# Autodesk Inventor assembly: 2016_IEEE_SouteastCon_Court v2
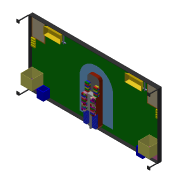
[picture p0: Inventor's stored thumbnail of the model, 180x180]
Saved by Autodesk Inventor 2015 (Build 190159000, 159)
## iProperties
Created: 2015-03-03
Part Number: 2016_IEEE_SouteastCon_Court v2
Document SubType Name: Assembly
Designer: Vukica
Author: Vukica
## Documents named in this file (17)
- C:\Users\Vukica\Dropbox\IEEE\hardware rules\2016Hardware_Court_v3\2016_IEEE_SouteastCon_Court v2.iam
- C:\Users\Vukica\Dropbox\IEEE\hardware rules\2016Hardware_Court\Base.ipt
- C:\Users\Vukica\Dropbox\IEEE\hardware rules\2016Hardware_Court\Ship area.ipt
- C:\Users\Vukica\Dropbox\IEEE\hardware rules\2016Hardware_Court\Starting position pink.ipt
- C:\Users\Vukica\Dropbox\IEEE\hardware rules\2016Hardware_Court\Starting position purple.ipt
- C:\Users\Vukica\Dropbox\IEEE\hardware rules\2016Hardware_Court\Rail zone.ipt
- C:\Users\Vukica\Dropbox\IEEE\hardware rules\2016Hardware_Court\Beacon.ipt
- C:\Users\Vukica\Dropbox\IEEE\hardware rules\2016Hardware_Court\Side 84 in by 6 in by half inch.ipt
- C:\Users\Vukica\Dropbox\IEEE\hardware rules\2016Hardware_Court\Side 120 in by 6 in by half inch.ipt
- C:\Users\Vukica\Dropbox\IEEE\hardware rules\2016Hardware_Court\Hill.ipt
- C:\Users\Vukica\Dropbox\IEEE\hardware rules\2016Hardware_Court\Blue truck.ipt
- C:\Users\Vukica\Dropbox\IEEE\hardware rules\2016Hardware_Court\Gold bar.ipt
- C:\Users\Vukica\Dropbox\IEEE\hardware rules\2016Hardware_Court\Tunnel.ipt
- C:\Users\Vukica\Dropbox\IEEE\hardware rules\2016Hardware_Court\Rail car.ipt
- C:\Users\Vukica\Dropbox\IEEE\hardware rules\2016Hardware_Court\Shipping goods QR subassembly.iam
- C:\Users\Vukica\Dropbox\IEEE\hardware rules\2016Hardware_Court\Shipping goods generic subassembly.iam
- C:\Users\Vukica\Dropbox\IEEE\hardware rules\2016Hardware_Court\Shipping goods colors subassembly.iam
## Components (36 placed, 16 different names)
1. Base:1 — Mate:1, Flush:1, Flush:2, Mate:2, Flush:3, Flush:4, Mate:3, Flush:5, Flush:6, Mate:4, Flush:7, Flush:8, Mate:5, Flush:9, Mate:7, Flush:11, Mate:9, Flush:12, Flush:13, Flush:15, Mate:10, Mate:11, Flush:16, Flush:18, Mate:12, Mate:17, Mate:22, Mate:30, Mate:38, Mate:40, Mate:43, Mate:46, Mate:53, Mate:55, Mate:62
2. Ship area:1 — Mate:1, Flush:1, Flush:2, Mate:6, Mate:49
3. Ship area:2 — Mate:2, Flush:3, Flush:4, Mate:8, Flush:10, Mate:54
4. Starting position pink:1 — Mate:4, Flush:7, Flush:8, Mate:64, Mate:88
5. Starting position purple:1 — Mate:3, Flush:5, Flush:6, Mate:89, Mate:105
6. Rail zone:1 — Mate:5, Mate:6, Flush:9, Mate:92, Flush:41
7. Rail zone:2 — Mate:7, Mate:8, Flush:10, Mate:90, Flush:40
8. Beacon:1 — Mate:14, Flush:22, Flush:23
9. Beacon:2 — Mate:13, Flush:20, Flush:21
10. Beacon:3 — Mate:15, Flush:24, Flush:25
11. Beacon:4 — Mate:16, Flush:26, Flush:27
12. Side 84 in by 6 in by half inch:1 — Mate:11, Flush:16, Flush:17, Mate:15, Flush:25, Mate:16, Flush:26, Flush:27, Mate:63, Flush:51
13. Side 84 in by 6 in by half inch:2 — Flush:18, Mate:12, Flush:19, Mate:13, Flush:21, Mate:14, Flush:23, Mate:39, Mate:41, Mate:44, Mate:47, Mate:106
14. Side 120 in by 6 in by half inch:1 — Flush:13, Flush:15, Mate:10, Flush:17, Flush:22, Flush:24, Mate:91, Mate:93
15. Side 120 in by 6 in by half inch:2 — Flush:11, Mate:9, Flush:12, Flush:19, Flush:20, Mate:23, Mate:32, Mate:84
16. Barge:1 — Mate:17, Mate:84, Mate:94, Flush:43, Flush:44, Mate:95, Flush:45, Flush:46, Mate:96, Mate:97, Flush:47, Mate:98, Flush:48, Mate:99, Mate:100, Flush:49, Mate:101, Mate:102, Flush:50, Mate:103, Flush:51
17. Blue truck:1 — Mate:22, Mate:23, Mate:89
18. Blue truck:2 — Mate:30, Mate:32, Mate:88
19. Gold bar:1 — Mate:38, Mate:39, Mate:42, Mate:45
20. Gold bar:2 — Mate:40, Mate:41, Mate:42, Mate:49
21. Gold bar:3 — Mate:43, Mate:44, Mate:45, Mate:48
22. Gold bar:4 — Mate:46, Mate:47, Mate:48
23. Gold bar:5 — Flush:30, Mate:50, Flush:31, Mate:51, Flush:32, Flush:33, Mate:53
24. Gold bar:6 — Flush:30, Mate:50, Flush:31, Mate:54, Mate:55
25. Gold bar:7 — Mate:51, Flush:32, Flush:33, Flush:34, Mate:52, Flush:35
26. Gold bar:8 — Flush:34, Mate:52, Flush:35
27. Tunnel:1 — Mate:62, Mate:63, Mate:64
28. Rail car:1 — Mate:90, Mate:91, Flush:40
29. Rail car:2 — Mate:92, Mate:93, Flush:41
30. Shipping goods QR subassembly:1 [sub-assembly] — Mate:94, Flush:43, Flush:44
31. Shipping goods QR subassembly:2 [sub-assembly] — Mate:95, Flush:45, Flush:46
32. Shipping goods generic subassembly:1 [sub-assembly] — Mate:96, Mate:97, Flush:47
33. Shipping goods generic subassembly:2 [sub-assembly] — Mate:98, Flush:48, Mate:99
34. Shipping goods colors subassembly:1 [sub-assembly] — Mate:102, Flush:50, Mate:103
35. Shipping goods colors subassembly:2 [sub-assembly] — Mate:100, Flush:49, Mate:101
36. Tunnel:2 — Mate:105, Mate:106
## Relationships (104: Mate 61, Flush 43)
- Mate:1: Base:1 ↔ Ship area:1
- Flush:1: Base:1 ↔ Ship area:1
- Flush:2: Base:1 ↔ Ship area:1
- Mate:2: Base:1 ↔ Ship area:2
- Flush:3: Base:1 ↔ Ship area:2
- Flush:4: Base:1 ↔ Ship area:2
- Mate:3: Base:1 ↔ Starting position purple:1
- Flush:5: Base:1 ↔ Starting position purple:1
- Flush:6: Base:1 ↔ Starting position purple:1
- Mate:4: Base:1 ↔ Starting position pink:1
- Flush:7: Base:1 ↔ Starting position pink:1
- Flush:8: Base:1 ↔ Starting position pink:1
- Mate:5: Base:1 ↔ Rail zone:1
- Mate:6: Ship area:1 ↔ Rail zone:1
- Flush:9: Base:1 ↔ Rail zone:1
- Mate:7: Base:1 ↔ Rail zone:2
- Mate:8: Ship area:2 ↔ Rail zone:2
- Flush:10: Ship area:2 ↔ Rail zone:2
- Flush:11: Base:1 ↔ Side 120 in by 6 in by half inch:2
- Mate:9: Base:1 ↔ Side 120 in by 6 in by half inch:2
- Flush:12: Base:1 ↔ Side 120 in by 6 in by half inch:2
- Flush:13: Base:1 ↔ Side 120 in by 6 in by half inch:1
- Flush:15: Base:1 ↔ Side 120 in by 6 in by half inch:1
- Mate:10: Base:1 ↔ Side 120 in by 6 in by half inch:1
- Mate:11: Base:1 ↔ Side 84 in by 6 in by half inch:1
- Flush:16: Base:1 ↔ Side 84 in by 6 in by half inch:1
- Flush:17: Side 84 in by 6 in by half inch:1 ↔ Side 120 in by 6 in by half inch:1
- Flush:18: Base:1 ↔ Side 84 in by 6 in by half inch:2
- Mate:12: Base:1 ↔ Side 84 in by 6 in by half inch:2
- Flush:19: Side 84 in by 6 in by half inch:2 ↔ Side 120 in by 6 in by half inch:2
- Mate:13: Beacon:2 ↔ Side 84 in by 6 in by half inch:2
- Flush:20: Beacon:2 ↔ Side 120 in by 6 in by half inch:2
- Flush:21: Beacon:2 ↔ Side 84 in by 6 in by half inch:2
- Mate:14: Beacon:1 ↔ Side 84 in by 6 in by half inch:2
- Flush:22: Beacon:1 ↔ Side 120 in by 6 in by half inch:1
- Flush:23: Beacon:1 ↔ Side 84 in by 6 in by half inch:2
- Mate:15: Beacon:3 ↔ Side 84 in by 6 in by half inch:1
- Flush:24: Beacon:3 ↔ Side 120 in by 6 in by half inch:1
- Flush:25: Beacon:3 ↔ Side 84 in by 6 in by half inch:1
- Mate:16: Beacon:4 ↔ Side 84 in by 6 in by half inch:1
- Flush:26: Beacon:4 ↔ Side 84 in by 6 in by half inch:1
- Flush:27: Beacon:4 ↔ Side 84 in by 6 in by half inch:1
- Mate:17: Base:1 ↔ Barge:1
- Mate:22: Base:1 ↔ Blue truck:1
- Mate:23: Side 120 in by 6 in by half inch:2 ↔ Blue truck:1
- Mate:30: Base:1 ↔ Blue truck:2
- Mate:32: Side 120 in by 6 in by half inch:2 ↔ Blue truck:2
- Mate:38: Base:1 ↔ Gold bar:1
- Mate:39: Side 84 in by 6 in by half inch:2 ↔ Gold bar:1
- Mate:40: Base:1 ↔ Gold bar:2
- Mate:41: Side 84 in by 6 in by half inch:2 ↔ Gold bar:2
- Mate:42: Gold bar:1 ↔ Gold bar:2
- Mate:43: Base:1 ↔ Gold bar:3
- Mate:44: Side 84 in by 6 in by half inch:2 ↔ Gold bar:3
- Mate:45: Gold bar:1 ↔ Gold bar:3
- Mate:46: Base:1 ↔ Gold bar:4
- Mate:47: Side 84 in by 6 in by half inch:2 ↔ Gold bar:4
- Mate:48: Gold bar:3 ↔ Gold bar:4
- Mate:49: Ship area:1 ↔ Gold bar:2
- Flush:30: Gold bar:5 ↔ Gold bar:6
- Mate:50: Gold bar:5 ↔ Gold bar:6
- Flush:31: Gold bar:5 ↔ Gold bar:6
- Mate:51: Gold bar:5 ↔ Gold bar:7
- Flush:32: Gold bar:5 ↔ Gold bar:7
- Flush:33: Gold bar:5 ↔ Gold bar:7
- Flush:34: Gold bar:7 ↔ Gold bar:8
- Mate:52: Gold bar:7 ↔ Gold bar:8
- Flush:35: Gold bar:7 ↔ Gold bar:8
- Mate:53: Base:1 ↔ Gold bar:5
- Mate:54: Ship area:2 ↔ Gold bar:6
- Mate:55: Base:1 ↔ Gold bar:6
- Mate:62: Base:1 ↔ Tunnel:1
- Mate:63: Side 84 in by 6 in by half inch:1 ↔ Tunnel:1
- Mate:64: Starting position pink:1 ↔ Tunnel:1
- Mate:84: Side 120 in by 6 in by half inch:2 ↔ Barge:1
- Mate:88: Starting position pink:1 ↔ Blue truck:2
- Mate:89: Starting position purple:1 ↔ Blue truck:1
- Mate:90: Rail zone:2 ↔ Rail car:1
- Mate:91 (50.8 mm): Side 120 in by 6 in by half inch:1 ↔ Rail car:1
- Flush:40: Rail zone:2 ↔ Rail car:1
- Mate:92: Rail zone:1 ↔ Rail car:2
- Mate:93 (50.8 mm): Side 120 in by 6 in by half inch:1 ↔ Rail car:2
- Flush:41: Rail zone:1 ↔ Rail car:2
- Mate:94: Barge:1 ↔ Shipping goods QR subassembly:1
- Flush:43: Barge:1 ↔ Shipping goods QR subassembly:1
- Flush:44: Barge:1 ↔ Shipping goods QR subassembly:1
- Mate:95: Barge:1 ↔ Shipping goods QR subassembly:2
- Flush:45: Barge:1 ↔ Shipping goods QR subassembly:2
- Flush:46: Barge:1 ↔ Shipping goods QR subassembly:2
- Mate:96: Barge:1 ↔ Shipping goods generic subassembly:1
- Mate:97: Barge:1 ↔ Shipping goods generic subassembly:1
- Flush:47: Barge:1 ↔ Shipping goods generic subassembly:1
- Mate:98: Barge:1 ↔ Shipping goods generic subassembly:2
- Flush:48: Barge:1 ↔ Shipping goods generic subassembly:2
- Mate:99: Barge:1 ↔ Shipping goods generic subassembly:2
- Mate:100: Barge:1 ↔ Shipping goods colors subassembly:2
- Flush:49: Barge:1 ↔ Shipping goods colors subassembly:2
- Mate:101: Barge:1 ↔ Shipping goods colors subassembly:2
- Mate:102: Barge:1 ↔ Shipping goods colors subassembly:1
- Flush:50: Barge:1 ↔ Shipping goods colors subassembly:1
- Mate:103: Barge:1 ↔ Shipping goods colors subassembly:1
- Mate:105: Starting position purple:1 ↔ Tunnel:2
- Mate:106: Side 84 in by 6 in by half inch:2 ↔ Tunnel:2
- Flush:51 (2209.8 mm): Side 84 in by 6 in by half inch:1 ↔ Barge:1
